# Autodesk Inventor assembly: złożenie
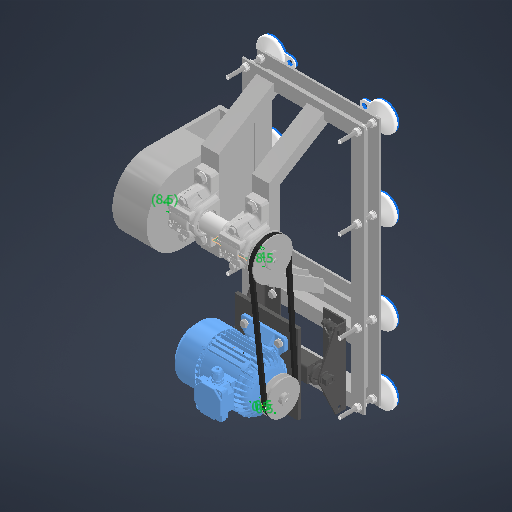
[picture p0: Inventor's stored thumbnail of the model, 512x512]
Saved by Autodesk Inventor 2026 (Build 300175050, 175E)
## iProperties
Created: 2025-06-02
Part Number: złożenie
Document SubType Name: Assembly
Designer: AdminForWorker
Title: złożenie v63
Author: AdminForWorker
## Documents named in this file (43)
- C:\Users\Public\Documents\Autodesk\Inventor 2026\złożenie.iam
- C:\Users\Public\Documents\Autodesk\Inventor 2026\kolo_pasowe_silnik v18.ipt
- C:\Users\Public\Documents\Autodesk\Inventor 2026\Sh80-.A v17.iam
- C:\Users\Public\Documents\Autodesk\Inventor 2026\obudowa wentylatora v4.ipt
- C:\Users\Public\Documents\Autodesk\Inventor 2026\System Naciągu pasa v3.ipt
- C:\Users\Public\Documents\Autodesk\Inventor 2026\pasklinowy v21.ipt
- C:\Users\Public\Documents\Autodesk\Inventor 2026\rama v27.ipt
- C:\Users\Public\Documents\Autodesk\Inventor 2026\kolo_pasowe_wiatrak v24.ipt
- C:\Users\Public\Documents\Autodesk\Inventor 2026\krazek_zabezpieczajacy_kolo_pasowe v3.ipt
- C:\Users\Public\Documents\Autodesk\Inventor 2026\Wpust A 8x7x25 v9.ipt
- C:\Users\Public\Documents\Autodesk\Inventor 2026\skf_bearing_1207_etn9_2 v5.iam
- C:\Users\Public\Documents\Autodesk\Inventor 2026\skf_bearing_1207_etn9_2 v5_1.iam
- C:\Users\Public\Documents\Autodesk\Inventor 2026\Podkładka Łożyskowa MB7 SKF v1.ipt
- C:\Users\Public\Documents\Autodesk\Inventor 2026\SKF_SNL 207 v7.iam
- C:\Users\Public\Documents\Autodesk\Inventor 2026\tuleja_kolo_pasowe v8.ipt
- C:\Users\Public\Documents\Autodesk\Inventor 2026\SKF_FRB 8_5_72 v1.ipt
- C:\Users\Public\Documents\Autodesk\Inventor 2026\SKF_SNL 207 v7_1.iam
- C:\Users\Public\Documents\Autodesk\Inventor 2026\Kołek walcowy 4m6x12 DIN 6325 v4.ipt
- C:\Users\Public\Documents\Autodesk\Inventor 2026\krazek_zabezpieczajacy_wentylator v3.ipt
- C:\Users\Public\Documents\Autodesk\Inventor 2026\tuleja_wiatrak v2.ipt
- C:\Users\Public\Documents\Autodesk\Inventor 2026\Podkładka PN-EN ISO 7089 - 10 Stal 100 HV Płaszczyzna v1.ipt
- C:\Users\Public\Documents\Autodesk\Inventor 2026\Podkładka PN-EN ISO 7089 - 14 Stal 100 HV Płaszczyzna v1.ipt
- C:\Users\Public\Documents\Autodesk\Inventor 2026\Podkładka PN-EN ISO 7089 - 5 Stal 100 HV Płaszczyzna v1.ipt
- C:\Users\Public\Documents\Autodesk\Inventor 2026\Wkręt z łbem sześciokątnym BS EN 24017 - M5 x 16 Stal 4.6 Płaszczyzna v1.ipt
- C:\Users\Public\Documents\Autodesk\Inventor 2026\Wkręt z łbem sześciokątnym PN-EN ISO 4017 - M14 x 50 Stal 4.6 Płaszczyzna v1.ipt
- C:\Users\Public\Documents\Autodesk\Inventor 2026\Wkręt z łbem sześciokątnym PN-EN ISO 4017 - M10 x 45 Stal 4.6 Płaszczyzna v1.ipt
- C:\Users\Public\Documents\Autodesk\Inventor 2026\Wkręt z łbem sześciokątnym PN-EN ISO 4017 - M10 x 35 Stal 4.6 Płaszczyzna v1.ipt
- C:\Users\Public\Documents\Autodesk\Inventor 2026\Nakrętka sześciokątna zwykła PN-EN ISO 4032 - M10 Stal 6 Płaszczyzna v1.ipt
- C:\Users\Public\Documents\Autodesk\Inventor 2026\Nakrętka sześciokątna zwykła PN-EN ISO 4032 - M14 Stal 6 Płaszczyzna v1.ipt
- C:\Users\Public\Documents\Autodesk\Inventor 2026\Wkręt z łbem sześciokątnym BS EN 24017 - M10 x 35 Stal 4.6 Płaszczyzna v1.ipt
- C:\Users\Public\Documents\Autodesk\Inventor 2026\SKF_TSN 207 A v1.ipt
- C:\Users\Public\Documents\Autodesk\Inventor 2026\27790-10-208010X1000 v3.ipt
- C:\Users\Public\Documents\Autodesk\Inventor 2026\Washer PN-EN ISO 7089 - 10 Steel 100 HV Plain v1.ipt
- C:\Users\Public\Documents\Autodesk\Inventor 2026\Hexagon Regular Nut ISO 4032 - M10 Steel 6 Plain v1.ipt
- C:\Users\Public\Documents\Autodesk\Inventor 2026\krążek zabezpieczający silnik v3.ipt
- C:\Users\Public\Documents\Autodesk\Inventor 2026\Washer PN-EN ISO 7089 - 4 Steel 100 HV Plain v1.ipt
- C:\Users\Public\Documents\Autodesk\Inventor 2026\Hexagon Head Screw BS EN 24017 - M4 x 10 Steel 4.6 Plain v1.ipt
- C:\Users\Public\Documents\Autodesk\Inventor 2026\Kołek walcowy 2m4x6 DIN 6325 v2.ipt
- C:\Users\Public\Documents\Autodesk\Inventor 2026\tuleja_silnik_1 v1.ipt
- C:\Users\Public\Documents\Autodesk\Inventor 2026\tuleja_silnik_2 v2.ipt
- C:\Users\Public\Documents\Autodesk\Inventor 2026\skf_nut_km_7_3D v1.ipt
- C:\Users\Public\Documents\Autodesk\Inventor 2026\Wał.ipt
- C:\Users\Salami\Downloads\item_0065496_śruba_z_łbem_walcowym_din_912_m3x10_szczegoły_3.ipt
## Components (145 placed, 40 different names)
1. kolo_pasowe_silnik v18:1 — Rotational:1
2. Sh80-.A v17:1 [sub-assembly]
3. obudowa wentylatora v4:1
4. System Naciągu pasa v3:1
5. pasklinowy v21:1 — Rotational:1
6. rama v27:1
7. kolo_pasowe_wiatrak v24:1
8. krazek_zabezpieczajacy_kolo_pasowe v3:1
9. Wpust A 8x7x25 v9:1 — Rotational:3
10. Wpust A 8x7x25 v9:2 — Rigid:1, Rigid:2
11. skf_bearing_1207_etn9_2 v5:1 [sub-assembly]
12. skf_bearing_1207_etn9_2 v5:2 [sub-assembly]
13. Podkładka Łożyskowa MB7 SKF v1:1
14. SKF_SNL 207 v7:1 [sub-assembly]
15. tuleja_kolo_pasowe v8:1
16. SKF_FRB 8_5_72 v1:1
17. SKF_FRB 8_5_72 v1:2
18. SKF_SNL 207 v7:2 [sub-assembly]
19. Kołek walcowy 4m6x12 DIN 6325 v4:1
20. krazek_zabezpieczajacy_wentylator v3:1 — Rotational:2
21. Kołek walcowy 4m6x12 DIN 6325 v4:2
22. tuleja_wiatrak v2:1
23. Podkładka PN-EN ISO 7089 - 10 Stal 100 HV Płaszczyzna v1:1
24. Podkładka PN-EN ISO 7089 - 10 Stal 100 HV Płaszczyzna v1:2
25. Podkładka PN-EN ISO 7089 - 10 Stal 100 HV Płaszczyzna v1:3
26. Podkładka PN-EN ISO 7089 - 10 Stal 100 HV Płaszczyzna v1:4
27. Podkładka PN-EN ISO 7089 - 10 Stal 100 HV Płaszczyzna v1:5
28. Podkładka PN-EN ISO 7089 - 10 Stal 100 HV Płaszczyzna v1:6
29. Podkładka PN-EN ISO 7089 - 10 Stal 100 HV Płaszczyzna v1:7
30. Podkładka PN-EN ISO 7089 - 10 Stal 100 HV Płaszczyzna v1:8
31. Podkładka PN-EN ISO 7089 - 14 Stal 100 HV Płaszczyzna v1:1
32. Podkładka PN-EN ISO 7089 - 14 Stal 100 HV Płaszczyzna v1:2
33. Podkładka PN-EN ISO 7089 - 14 Stal 100 HV Płaszczyzna v1:3
34. Podkładka PN-EN ISO 7089 - 14 Stal 100 HV Płaszczyzna v1:4
35. Podkładka PN-EN ISO 7089 - 5 Stal 100 HV Płaszczyzna v1:1
36. Podkładka PN-EN ISO 7089 - 5 Stal 100 HV Płaszczyzna v1:2
37. Wkręt z łbem sześciokątnym BS EN 24017 - M5 x 16 Stal 4.6 Płaszczyzna v1:1
38. Wkręt z łbem sześciokątnym BS EN 24017 - M5 x 16 Stal 4.6 Płaszczyzna v1:2
39. Wkręt z łbem sześciokątnym PN-EN ISO 4017 - M14 x 50 Stal 4.6 Płaszczyzna v1:1
40. Wkręt z łbem sześciokątnym PN-EN ISO 4017 - M14 x 50 Stal 4.6 Płaszczyzna v1:2
41. Wkręt z łbem sześciokątnym PN-EN ISO 4017 - M14 x 50 Stal 4.6 Płaszczyzna v1:3 — Symmetry:1
42. Wkręt z łbem sześciokątnym PN-EN ISO 4017 - M14 x 50 Stal 4.6 Płaszczyzna v1:4 — Symmetry:1
43. Wkręt z łbem sześciokątnym PN-EN ISO 4017 - M10 x 45 Stal 4.6 Płaszczyzna v1:3
44. Wkręt z łbem sześciokątnym PN-EN ISO 4017 - M10 x 45 Stal 4.6 Płaszczyzna v1:4
45. Wkręt z łbem sześciokątnym PN-EN ISO 4017 - M10 x 45 Stal 4.6 Płaszczyzna v1:5
46. Wkręt z łbem sześciokątnym PN-EN ISO 4017 - M10 x 45 Stal 4.6 Płaszczyzna v1:6
47. Wkręt z łbem sześciokątnym PN-EN ISO 4017 - M10 x 45 Stal 4.6 Płaszczyzna v1:1
48. Wkręt z łbem sześciokątnym PN-EN ISO 4017 - M10 x 35 Stal 4.6 Płaszczyzna v1:1
49. Podkładka PN-EN ISO 7089 - 14 Stal 100 HV Płaszczyzna v1:5
50. Podkładka PN-EN ISO 7089 - 14 Stal 100 HV Płaszczyzna v1:6
51. Podkładka PN-EN ISO 7089 - 14 Stal 100 HV Płaszczyzna v1:7
52. Podkładka PN-EN ISO 7089 - 14 Stal 100 HV Płaszczyzna v1:8
53. Podkładka PN-EN ISO 7089 - 10 Stal 100 HV Płaszczyzna v1:9
54. Podkładka PN-EN ISO 7089 - 10 Stal 100 HV Płaszczyzna v1:10
55. Podkładka PN-EN ISO 7089 - 10 Stal 100 HV Płaszczyzna v1:11
56. Podkładka PN-EN ISO 7089 - 10 Stal 100 HV Płaszczyzna v1:12
57. Podkładka PN-EN ISO 7089 - 10 Stal 100 HV Płaszczyzna v1:13
58. Podkładka PN-EN ISO 7089 - 10 Stal 100 HV Płaszczyzna v1:14
59. Nakrętka sześciokątna zwykła PN-EN ISO 4032 - M10 Stal 6 Płaszczyzna v1:1
60. Nakrętka sześciokątna zwykła PN-EN ISO 4032 - M10 Stal 6 Płaszczyzna v1:2
61. Nakrętka sześciokątna zwykła PN-EN ISO 4032 - M10 Stal 6 Płaszczyzna v1:3
62. Nakrętka sześciokątna zwykła PN-EN ISO 4032 - M10 Stal 6 Płaszczyzna v1:4
63. Nakrętka sześciokątna zwykła PN-EN ISO 4032 - M10 Stal 6 Płaszczyzna v1:5
64. Nakrętka sześciokątna zwykła PN-EN ISO 4032 - M10 Stal 6 Płaszczyzna v1:6
65. Nakrętka sześciokątna zwykła PN-EN ISO 4032 - M14 Stal 6 Płaszczyzna v1:1
66. Nakrętka sześciokątna zwykła PN-EN ISO 4032 - M14 Stal 6 Płaszczyzna v1:2
67. Nakrętka sześciokątna zwykła PN-EN ISO 4032 - M14 Stal 6 Płaszczyzna v1:3
68. Nakrętka sześciokątna zwykła PN-EN ISO 4032 - M14 Stal 6 Płaszczyzna v1:4
69. Wkręt z łbem sześciokątnym BS EN 24017 - M10 x 35 Stal 4.6 Płaszczyzna v1:1
70. Wkręt z łbem sześciokątnym BS EN 24017 - M10 x 35 Stal 4.6 Płaszczyzna v1:2
71. Podkładka PN-EN ISO 7089 - 10 Stal 100 HV Płaszczyzna v1:15
72. Podkładka PN-EN ISO 7089 - 10 Stal 100 HV Płaszczyzna v1:16
73. Nakrętka sześciokątna zwykła PN-EN ISO 4032 - M10 Stal 6 Płaszczyzna v1:7
74. Nakrętka sześciokątna zwykła PN-EN ISO 4032 - M10 Stal 6 Płaszczyzna v1:8
75. SKF_TSN 207 A v1:2
76. SKF_TSN 207 A v1:3
77. SKF_TSN 207 A v1:4
78. SKF_TSN 207 A v1:5
79. 27790-10-208010X1000 v3:1
80. 27790-10-208010X1000 v3:2
81. 27790-10-208010X1000 v3:3
82. 27790-10-208010X1000 v3:4
83. 27790-10-208010X1000 v3:5
84. 27790-10-208010X1000 v3:6
85. 27790-10-208010X1000 v3:7
86. 27790-10-208010X1000 v3:8
87. Washer PN-EN ISO 7089 - 10 Steel 100 HV Plain v1:1
88. Washer PN-EN ISO 7089 - 10 Steel 100 HV Plain v1:2
89. Washer PN-EN ISO 7089 - 10 Steel 100 HV Plain v1:3
90. Washer PN-EN ISO 7089 - 10 Steel 100 HV Plain v1:4
91. Washer PN-EN ISO 7089 - 10 Steel 100 HV Plain v1:5
92. Washer PN-EN ISO 7089 - 10 Steel 100 HV Plain v1:6
93. Washer PN-EN ISO 7089 - 10 Steel 100 HV Plain v1:7
94. Washer PN-EN ISO 7089 - 10 Steel 100 HV Plain v1:8
95. Washer PN-EN ISO 7089 - 10 Steel 100 HV Plain v1:9
96. Washer PN-EN ISO 7089 - 10 Steel 100 HV Plain v1:10
97. Washer PN-EN ISO 7089 - 10 Steel 100 HV Plain v1:11
98. Washer PN-EN ISO 7089 - 10 Steel 100 HV Plain v1:12
99. Washer PN-EN ISO 7089 - 10 Steel 100 HV Plain v1:13
100. Washer PN-EN ISO 7089 - 10 Steel 100 HV Plain v1:14
101. Washer PN-EN ISO 7089 - 10 Steel 100 HV Plain v1:15
102. Washer PN-EN ISO 7089 - 10 Steel 100 HV Plain v1:16
103. Washer PN-EN ISO 7089 - 10 Steel 100 HV Plain v1:17
104. Washer PN-EN ISO 7089 - 10 Steel 100 HV Plain v1:18
105. Washer PN-EN ISO 7089 - 10 Steel 100 HV Plain v1:19
106. Washer PN-EN ISO 7089 - 10 Steel 100 HV Plain v1:20
107. Washer PN-EN ISO 7089 - 10 Steel 100 HV Plain v1:21
108. Washer PN-EN ISO 7089 - 10 Steel 100 HV Plain v1:22
109. Washer PN-EN ISO 7089 - 10 Steel 100 HV Plain v1:23
110. Washer PN-EN ISO 7089 - 10 Steel 100 HV Plain v1:24
111. Hexagon Regular Nut ISO 4032 - M10 Steel 6 Plain v1:1
112. Hexagon Regular Nut ISO 4032 - M10 Steel 6 Plain v1:2
113. Hexagon Regular Nut ISO 4032 - M10 Steel 6 Plain v1:3
114. Hexagon Regular Nut ISO 4032 - M10 Steel 6 Plain v1:4
115. Hexagon Regular Nut ISO 4032 - M10 Steel 6 Plain v1:5
116. Hexagon Regular Nut ISO 4032 - M10 Steel 6 Plain v1:6
117. Hexagon Regular Nut ISO 4032 - M10 Steel 6 Plain v1:7
118. Hexagon Regular Nut ISO 4032 - M10 Steel 6 Plain v1:8
119. Hexagon Regular Nut ISO 4032 - M10 Steel 6 Plain v1:9
120. Hexagon Regular Nut ISO 4032 - M10 Steel 6 Plain v1:10
121. Hexagon Regular Nut ISO 4032 - M10 Steel 6 Plain v1:11
122. Hexagon Regular Nut ISO 4032 - M10 Steel 6 Plain v1:12
123. Hexagon Regular Nut ISO 4032 - M10 Steel 6 Plain v1:13
124. Hexagon Regular Nut ISO 4032 - M10 Steel 6 Plain v1:14
125. Hexagon Regular Nut ISO 4032 - M10 Steel 6 Plain v1:15
126. Hexagon Regular Nut ISO 4032 - M10 Steel 6 Plain v1:16
127. Hexagon Regular Nut ISO 4032 - M10 Steel 6 Plain v1:17
128. Hexagon Regular Nut ISO 4032 - M10 Steel 6 Plain v1:18
129. Hexagon Regular Nut ISO 4032 - M10 Steel 6 Plain v1:19
130. Hexagon Regular Nut ISO 4032 - M10 Steel 6 Plain v1:20
131. Hexagon Regular Nut ISO 4032 - M10 Steel 6 Plain v1:21
132. Hexagon Regular Nut ISO 4032 - M10 Steel 6 Plain v1:22
133. Hexagon Regular Nut ISO 4032 - M10 Steel 6 Plain v1:23
134. Hexagon Regular Nut ISO 4032 - M10 Steel 6 Plain v1:24
135. krążek zabezpieczający silnik v3:1
136. Washer PN-EN ISO 7089 - 4 Steel 100 HV Plain v1:1
137. Hexagon Head Screw BS EN 24017 - M4 x 10 Steel 4.6 Plain v1:1
138. Kołek walcowy 2m4x6 DIN 6325 v2:1
139. tuleja_silnik_1 v1:1
140. tuleja_silnik_2 v2:1
141. skf_nut_km_7_3D v1:2
142. Wał:1 — Rotational:2, Rigid:1
143. item_0065496_śruba_z_łbem_walcowym_din_912_m3x10_szczegoły_3:1 — Rigid:2
144. item_0065496_śruba_z_łbem_walcowym_din_912_m3x10_szczegoły_3:2
145. item_0065496_śruba_z_łbem_walcowym_din_912_m3x10_szczegoły_3:4 — Rotational:3
## Relationships (6: RevoluteJoint 3, WeldJoint 2, Symmetry 1)
- Symmetry:1: Wkręt z łbem sześciokątnym PN-EN ISO 4017 - M14 x 50 Stal 4.6 Płaszczyzna v1:3 ↔ Wkręt z łbem sześciokątnym PN-EN ISO 4017 - M14 x 50 Stal 4.6 Płaszczyzna v1:4
- Rotational:1 [RevoluteJoint]: kolo_pasowe_silnik v18:1 ↔ pasklinowy v21:1
- Rotational:2 [RevoluteJoint]: krazek_zabezpieczajacy_wentylator v3:1 ↔ Wał:1
- Rigid:1 [WeldJoint]: Wpust A 8x7x25 v9:2 ↔ Wał:1
- Rigid:2 [WeldJoint]: Wpust A 8x7x25 v9:2 ↔ item_0065496_śruba_z_łbem_walcowym_din_912_m3x10_szczegoły_3:1
- Rotational:3 [RevoluteJoint]: Wpust A 8x7x25 v9:1 ↔ item_0065496_śruba_z_łbem_walcowym_din_912_m3x10_szczegoły_3:4
